# Autodesk Inventor assembly: Drivetrain
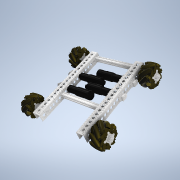
[picture p0: Inventor's stored thumbnail of the model, 180x180]
Saved by Autodesk Inventor 2020 (Build 240168000, 168)
## iProperties
Created: 2020-09-22
Part Number: Drivetrain
Document SubType Name: Assembly
Designer: tdmp4
Author: tdmp4
## Documents named in this file (13)
- C:\Users\tdmp4\Documents\GitHub\CAD-2021-Ultimate_Goal\Drivetrain\Drivetrain.iam
- C:\Users\tdmp4\Documents\GitHub\CAD-2021-Ultimate_Goal\ServoCity\585460.ipt
- C:\Users\tdmp4\Documents\GitHub\CAD-2021-Ultimate_Goal\GoBilda\1206-0016-0004 assembly.ipt
- C:\Users\tdmp4\Documents\GitHub\CAD-2021-Ultimate_Goal\GoBilda\5202-0002-0014 part.ipt
- C:\Users\tdmp4\Documents\GitHub\CAD-2021-Ultimate_Goal\ServoCity\625051 assembly.ipt
- C:\Users\tdmp4\Documents\GitHub\CAD-2021-Ultimate_Goal\ServoCity\634064.ipt
- C:\Users\tdmp4\Documents\GitHub\CAD-2021-Ultimate_Goal\ServoCity\545619 assembly.ipt
- C:\Users\tdmp4\Documents\GitHub\CAD-2021-Ultimate_Goal\ServoCity\535198.ipt
- C:\Users\tdmp4\Documents\GitHub\CAD-2021-Ultimate_Goal\ServoCity\615102.ipt
- C:\Users\tdmp4\Documents\GitHub\CAD-2021-Ultimate_Goal\Drivetrain\FrontR_BackL_MecW.iam
- C:\Users\tdmp4\Documents\GitHub\CAD-2021-Ultimate_Goal\ServoCity\7in-Xrail.ipt
- C:\Users\tdmp4\Documents\GitHub\CAD-2021-Ultimate_Goal\Drivetrain\FrontL_BackR_MecW.iam
- C:\Users\tdmp4\Documents\GitHub\CAD-2021-Ultimate_Goal\ServoCity\634082.ipt
## Components (52 placed, 13 different names)
1. 585460:1 — Mate:40, Mate:41, Mate:42, Mate:43, Mate:44, Mate:45, Mate:53, Mate:55, Mate:60, Mate:61, Mate:62, Mate:63, Mate:64, Mate:65, Flush:3, Mate:68, Mate:78, Mate:79, Mate:80, Mate:89, Mate:90, Mate:91, Mate:96, Mate:97, Mate:98, Mate:99, Mate:100, Mate:101, Mate:103, Mate:105, Mate:130, Mate:131, Mate:132, Mate:133, Mate:135, Mate:136
2. 585460:2 — Mate:10, Mate:11, Mate:12, Mate:16, Mate:17, Mate:23, Mate:24, Mate:25, Mate:26, Mate:27, Mate:28, Flush:2, Mate:30, Mate:33, Mate:37, Mate:38, Mate:39, Mate:72, Mate:73, Mate:74, Mate:106, Mate:107, Mate:108, Mate:109, Mate:110, Mate:111, Mate:116, Mate:117, Mate:118, Flush:4, Mate:124, Mate:126, Mate:127, Mate:128, Mate:129, Mate:134
3. 1206-0016-0004 assembly:1 — Mate:10, Mate:11, Mate:12, Mate:13, Mate:14, Mate:15
4. 1206-0016-0004 assembly:2 — Mate:43, Mate:44, Mate:45, Mate:46, Mate:47, Mate:48
5. 5202-0002-0014 part:1 — Mate:81, Mate:82, Mate:83, Mate:84, Mate:85, Mate:86, Mate:88
6. 5202-0002-0014 part:2 — Mate:46, Mate:47, Mate:48, Mate:49, Mate:50, Mate:52
7. 5202-0002-0014 part:3 — Mate:75, Mate:76, Mate:77, Mate:112, Mate:113, Mate:114
8. 5202-0002-0014 part:4 — Mate:7, Flush:1, Mate:9, Mate:13, Mate:14, Mate:15
9. 625051 assembly:1 — Mate:112, Mate:113, Mate:115
10. 625051 assembly:2 — Mate:85, Mate:86, Mate:87
11. 625051 assembly:3 — Mate:49, Mate:50, Mate:51
12. 625051 assembly:4 — Mate:7, Flush:1, Mate:8
13. 634064:1 — Mate:51, Mate:52, Mate:54, Mate:56, Mate:58
14. 634064:2 — Mate:87, Mate:88, Mate:92, Mate:94
15. 634064:3 — Mate:8, Mate:9, Mate:32, Mate:35
16. 634064:4 — Mate:114, Mate:115, Mate:119, Mate:121
17. 545619 assembly:1 — Mate:99, Mate:100, Mate:101
18. 545619 assembly:2 — Mate:106, Mate:107, Mate:108, Mate:123
19. 545619 assembly:3 — Mate:120, Mate:121, Mate:122
20. 545619 assembly:4 — Mate:109, Mate:110, Mate:111
21. 545619 assembly:6 — Mate:93, Mate:94, Mate:95
22. 545619 assembly:8 — Mate:60, Mate:61, Mate:62
23. 545619 assembly:9 — Mate:57, Mate:58, Mate:59
24. 545619 assembly:10 — Mate:96, Mate:97, Mate:98, Mate:102
25. 545619 assembly:13 — Mate:63, Mate:64, Mate:65, Mate:66
26. 545619 assembly:14 — Mate:23, Mate:24, Mate:25, Mate:29
27. 545619 assembly:15 — Mate:26, Mate:27, Mate:28
28. 545619 assembly:16 — Mate:34, Mate:35, Mate:36
29. 535198:1 — Mate:126, Mate:127
30. 535198:2 — Mate:89, Mate:90
31. 535198:6 — Mate:116, Mate:117
32. 535198:7 — Mate:128, Mate:129
33. 535198:8 — Mate:132, Mate:133
34. 535198:13 — Mate:130, Mate:131
35. 535198:18 — Mate:53, Mate:54
36. 535198:19 — Mate:16, Mate:17
37. 615102:1 — Mate:32, Mate:33, Mate:34, Mate:36
38. 615102:6 — Mate:91, Mate:92, Mate:93, Mate:95
39. 615102:7 — Mate:118, Mate:119, Mate:120, Mate:122
40. 615102:8 — Mate:55, Mate:56, Mate:57, Mate:59
41. 634082:1 — Mate:123, Flush:4, Mate:125
42. 634082:2 — Mate:29, Flush:2, Mate:31
43. 634082:3 — Mate:102, Mate:103, Mate:104
44. 634082:4 — Mate:66, Flush:3, Mate:67
45. FrontR_BackL_MecW:1 [sub-assembly] — Mate:30, Mate:31
46. FrontR_BackL_MecW:2 [sub-assembly] — Mate:104, Mate:105
47. 7in-Xrail:1 — Mate:37, Mate:38, Mate:39, Mate:40, Mate:41, Mate:42
48. mmm — Mate:134, Mate:135, Mate:136
49. FrontL_BackR_MecW:1 [sub-assembly] — Mate:67, Mate:68
50. FrontL_BackR_MecW:2 [sub-assembly] — Mate:124, Mate:125
51. 1206-0016-0004 assembly:3 — Mate:72, Mate:73, Mate:74, Mate:75, Mate:76, Mate:77
52. 1206-0016-0004 assembly:4 — Mate:78, Mate:79, Mate:80, Mate:81, Mate:82, Mate:83, Mate:84
## Relationships (126: Mate 122, Flush 4)
- Mate:7: 5202-0002-0014 part:4 ↔ 625051 assembly:4
- Flush:1: 5202-0002-0014 part:4 ↔ 625051 assembly:4
- Mate:8: 625051 assembly:4 ↔ 634064:3
- Mate:9: 5202-0002-0014 part:4 ↔ 634064:3
- Mate:10: 585460:2 ↔ 1206-0016-0004 assembly:1
- Mate:11: 585460:2 ↔ 1206-0016-0004 assembly:1
- Mate:12: 585460:2 ↔ 1206-0016-0004 assembly:1
- Mate:13: 1206-0016-0004 assembly:1 ↔ 5202-0002-0014 part:4
- Mate:14: 1206-0016-0004 assembly:1 ↔ 5202-0002-0014 part:4
- Mate:15: 1206-0016-0004 assembly:1 ↔ 5202-0002-0014 part:4
- Mate:16: 585460:2 ↔ 535198:19
- Mate:17: 585460:2 ↔ 535198:19
- Mate:23: 585460:2 ↔ 545619 assembly:14
- Mate:24: 585460:2 ↔ 545619 assembly:14
- Mate:25: 585460:2 ↔ 545619 assembly:14
- Mate:26: 585460:2 ↔ 545619 assembly:15
- Mate:27: 585460:2 ↔ 545619 assembly:15
- Mate:28: 585460:2 ↔ 545619 assembly:15
- Mate:29: 545619 assembly:14 ↔ 634082:2
- Flush:2: 585460:2 ↔ 634082:2
- Mate:30 (3.81 mm): 585460:2 ↔ FrontR_BackL_MecW:1
- Mate:31: 634082:2 ↔ FrontR_BackL_MecW:1
- Mate:32: 634064:3 ↔ 615102:1
- Mate:33 (3.81 mm): 585460:2 ↔ 615102:1
- Mate:34 (5.08 mm): 545619 assembly:16 ↔ 615102:1
- Mate:35: 634064:3 ↔ 545619 assembly:16
- Mate:36: 545619 assembly:16 ↔ 615102:1
- Mate:37: 585460:2 ↔ 7in-Xrail:1
- Mate:38: 585460:2 ↔ 7in-Xrail:1
- Mate:39: 585460:2 ↔ 7in-Xrail:1
- Mate:40: 585460:1 ↔ 7in-Xrail:1
- Mate:41: 585460:1 ↔ 7in-Xrail:1
- Mate:42: 585460:1 ↔ 7in-Xrail:1
- Mate:43: 585460:1 ↔ 1206-0016-0004 assembly:2
- Mate:44: 585460:1 ↔ 1206-0016-0004 assembly:2
- Mate:45: 585460:1 ↔ 1206-0016-0004 assembly:2
- Mate:46: 1206-0016-0004 assembly:2 ↔ 5202-0002-0014 part:2
- Mate:47: 1206-0016-0004 assembly:2 ↔ 5202-0002-0014 part:2
- Mate:48: 1206-0016-0004 assembly:2 ↔ 5202-0002-0014 part:2
- Mate:49: 5202-0002-0014 part:2 ↔ 625051 assembly:3
- Mate:50: 5202-0002-0014 part:2 ↔ 625051 assembly:3
- Mate:51: 625051 assembly:3 ↔ 634064:1
- Mate:52: 5202-0002-0014 part:2 ↔ 634064:1
- Mate:53: 585460:1 ↔ 535198:18
- Mate:54: 634064:1 ↔ 535198:18
- Mate:55 (3.81 mm): 585460:1 ↔ 615102:8
- Mate:56: 634064:1 ↔ 615102:8
- Mate:57 (5.08 mm): 545619 assembly:9 ↔ 615102:8
- Mate:58: 634064:1 ↔ 545619 assembly:9
- Mate:59: 545619 assembly:9 ↔ 615102:8
- Mate:60: 585460:1 ↔ 545619 assembly:8
- Mate:61: 585460:1 ↔ 545619 assembly:8
- Mate:62: 585460:1 ↔ 545619 assembly:8
- Mate:63: 585460:1 ↔ 545619 assembly:13
- Mate:64: 585460:1 ↔ 545619 assembly:13
- Mate:65: 585460:1 ↔ 545619 assembly:13
- Mate:66: 545619 assembly:13 ↔ 634082:4
- Flush:3 (-25.4 mm): 585460:1 ↔ 634082:4
- Mate:67: 634082:4 ↔ FrontL_BackR_MecW:1
- Mate:68 (5.08 mm): 585460:1 ↔ FrontL_BackR_MecW:1
- Mate:72: 585460:2 ↔ 1206-0016-0004 assembly:3
- Mate:73: 585460:2 ↔ 1206-0016-0004 assembly:3
- Mate:74: 585460:2 ↔ 1206-0016-0004 assembly:3
- Mate:75: 5202-0002-0014 part:3 ↔ 1206-0016-0004 assembly:3
- Mate:76: 5202-0002-0014 part:3 ↔ 1206-0016-0004 assembly:3
- Mate:77: 5202-0002-0014 part:3 ↔ 1206-0016-0004 assembly:3
- Mate:78: 585460:1 ↔ 1206-0016-0004 assembly:4
- Mate:79: 585460:1 ↔ 1206-0016-0004 assembly:4
- Mate:80: 585460:1 ↔ 1206-0016-0004 assembly:4
- Mate:81: 5202-0002-0014 part:1 ↔ 1206-0016-0004 assembly:4
- Mate:82: 5202-0002-0014 part:1 ↔ 1206-0016-0004 assembly:4
- Mate:83: 5202-0002-0014 part:1 ↔ 1206-0016-0004 assembly:4
- Mate:84: 5202-0002-0014 part:1 ↔ 1206-0016-0004 assembly:4
- Mate:85: 5202-0002-0014 part:1 ↔ 625051 assembly:2
- Mate:86: 5202-0002-0014 part:1 ↔ 625051 assembly:2
- Mate:87: 625051 assembly:2 ↔ 634064:2
- Mate:88: 5202-0002-0014 part:1 ↔ 634064:2
- Mate:89: 585460:1 ↔ 535198:2
- Mate:90: 585460:1 ↔ 535198:2
- Mate:91 (3.81 mm): 585460:1 ↔ 615102:6
- Mate:92: 634064:2 ↔ 615102:6
- Mate:93 (5.08 mm): 545619 assembly:6 ↔ 615102:6
- Mate:94: 634064:2 ↔ 545619 assembly:6
- Mate:95: 545619 assembly:6 ↔ 615102:6
- Mate:96: 585460:1 ↔ 545619 assembly:10
- Mate:97: 585460:1 ↔ 545619 assembly:10
- Mate:98: 585460:1 ↔ 545619 assembly:10
- Mate:99: 585460:1 ↔ 545619 assembly:1
- Mate:100: 585460:1 ↔ 545619 assembly:1
- Mate:101: 585460:1 ↔ 545619 assembly:1
- Mate:102: 545619 assembly:10 ↔ 634082:3
- Mate:103 (25.4 mm): 585460:1 ↔ 634082:3
- Mate:104: 634082:3 ↔ FrontR_BackL_MecW:2
- Mate:105 (3.81 mm): 585460:1 ↔ FrontR_BackL_MecW:2
- Mate:106: 585460:2 ↔ 545619 assembly:2
- Mate:107: 585460:2 ↔ 545619 assembly:2
- Mate:108: 585460:2 ↔ 545619 assembly:2
- Mate:109: 585460:2 ↔ 545619 assembly:4
- Mate:110: 585460:2 ↔ 545619 assembly:4
- Mate:111: 585460:2 ↔ 545619 assembly:4
- Mate:112: 5202-0002-0014 part:3 ↔ 625051 assembly:1
- Mate:113: 5202-0002-0014 part:3 ↔ 625051 assembly:1
- Mate:114: 5202-0002-0014 part:3 ↔ 634064:4
- Mate:115: 625051 assembly:1 ↔ 634064:4
- Mate:116: 585460:2 ↔ 535198:6
- Mate:117: 585460:2 ↔ 535198:6
- Mate:118 (3.81 mm): 585460:2 ↔ 615102:7
- Mate:119: 634064:4 ↔ 615102:7
- Mate:120 (5.08 mm): 545619 assembly:3 ↔ 615102:7
- Mate:121: 634064:4 ↔ 545619 assembly:3
- Mate:122: 545619 assembly:3 ↔ 615102:7
- Mate:123: 545619 assembly:2 ↔ 634082:1
- Flush:4: 585460:2 ↔ 634082:1
- Mate:124 (3.81 mm): 585460:2 ↔ FrontL_BackR_MecW:2
- Mate:125: 634082:1 ↔ FrontL_BackR_MecW:2
- Mate:126: 585460:2 ↔ 535198:1
- Mate:127: 585460:2 ↔ 535198:1
- Mate:128: 585460:2 ↔ 535198:7
- Mate:129: 585460:2 ↔ 535198:7
- Mate:130: 585460:1 ↔ 535198:13
- Mate:131: 585460:1 ↔ 535198:13
- Mate:132: 585460:1 ↔ 535198:8
- Mate:133: 585460:1 ↔ 535198:8
- Mate:134: 585460:2 ↔ mmm
- Mate:135: 585460:1 ↔ mmm
- Mate:136: 585460:1 ↔ mmm
